# Autodesk Inventor assembly: YflanecSborka
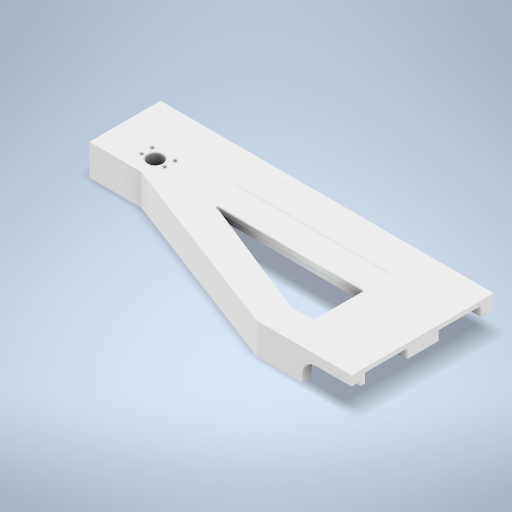
[picture p0: Inventor's stored thumbnail of the model, 512x512]
Saved by Autodesk Inventor 2024 (Build 280153000, 153)
## iProperties
Created: 2023-06-18
Part Number: YflanecSborka
Document SubType Name: Assembly
Designer: KirikDK
Author: KirikDK
## Documents named in this file (5)
- C:\Users\KirikDK\Documents\Stanok2023\YflanecSborka.iam
- C:\Users\KirikDK\Documents\Stanok2023\YFlanPlate.ipt
- C:\Users\KirikDK\Documents\Stanok2023\PortalFlanec.ipt
- C:\Users\KirikDK\Documents\Stanok2023\YflanecYcrepA.ipt
- C:\Users\KirikDK\Documents\Stanok2023\Y_zigZag.ipt
## Components (4 placed, 4 different names)
1. YFlanPlate:1 — Mate:1, Flush:1, Flush:2, Flush:4, Mate:3, Flush:5
2. PortalFlanec:1 — Mate:1, Flush:1, Flush:2, Mate:2, Flush:3, Flush:6
3. YflanecYcrepA:1 — Mate:2, Flush:3, Flush:4
4. Y_zigZag:2 — Mate:3, Flush:5, Flush:6
## Relationships (9: Flush 6, Mate 3)
- Mate:1: YFlanPlate:1 ↔ PortalFlanec:1
- Flush:1: YFlanPlate:1 ↔ PortalFlanec:1
- Flush:2: YFlanPlate:1 ↔ PortalFlanec:1
- Mate:2: PortalFlanec:1 ↔ YflanecYcrepA:1
- Flush:3: PortalFlanec:1 ↔ YflanecYcrepA:1
- Flush:4: YFlanPlate:1 ↔ YflanecYcrepA:1
- Mate:3: YFlanPlate:1 ↔ Y_zigZag:2
- Flush:5: YFlanPlate:1 ↔ Y_zigZag:2
- Flush:6: PortalFlanec:1 ↔ Y_zigZag:2
